# Autodesk Inventor assembly: pre camera mount assem
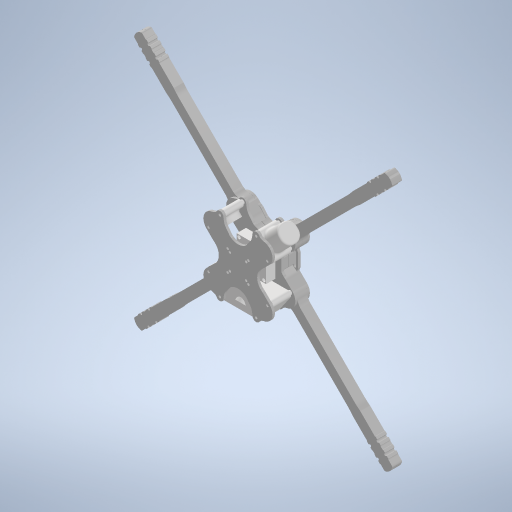
[picture p0: Inventor's stored thumbnail of the model, 512x512]
Saved by Autodesk Inventor 2023 (Build 270158000, 158)
## iProperties
Created: 2023-01-23
Part Number: pre camera mount assem
Document SubType Name: Assembly
Designer: Steven
Author: Steven
## Documents named in this file (3)
- Y:\FPV drone stuff\0 Street League\Frames\experimental-quad-frames\Nightstick MAX\3D prints\assems for derivs\pre camera mount assem.iam
- Y:\FPV drone stuff\0 Street League\Frames\experimental-quad-frames\Nightstick MAX\NightStickmax full assem.iam
- Y:\FPV drone stuff\0 Street League\Frames\experimental-quad-frames\Nightstick MAX\3D prints\assems for derivs\pre camera mount block.ipt
## Components (2 placed, 2 different names)
1. NightStickmax full assem:1 [sub-assembly] — Flush:1, Flush:2, Flush:3, Mate:1, Mate:2, Flush:4
2. pre camera mount block:1 — Mate:1, Mate:2, Flush:4
## Relationships (6: Flush 4, Mate 2)
- Flush:1: NightStickmax full assem:1
- Flush:2: NightStickmax full assem:1
- Flush:3: NightStickmax full assem:1
- Mate:1: NightStickmax full assem:1 ↔ pre camera mount block:1
- Mate:2: NightStickmax full assem:1 ↔ pre camera mount block:1
- Flush:4: NightStickmax full assem:1 ↔ pre camera mount block:1
